# Autodesk Inventor assembly: basicLift
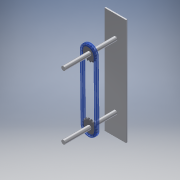
[picture p0: Inventor's stored thumbnail of the model, 180x180]
Saved by Autodesk Inventor 2016 SP1 (Build 200210100, 210)
## iProperties
Created: 2016-02-01
Part Number: basicLift
Document SubType Name: Assembly
Designer: steele
Mass: 210.898 g
Surface Area: 537.048 cm^2
Volume: 77.5037 cm^3
Density: 2.72113 g/cm^3
Author: steele
## Documents named in this file (4)
- C:\snobotics\CAD-Development\robSteele\SnoBotics2016\2016-01-31-Lift\basicLift.iam
- C:\snobotics\CAD-Development\robSteele\SnoBotics2016\2016-01-31-Lift\basicLiftPlate.ipt
- C:\snobotics\CAD-Development\robSteele\SnoBotics2016\2016-01-31-Lift\basicLeftAxel.ipt
- C:\snobotics\CAD-Development\robSteele\SnoBotics2016\2016-01-31-Lift\basicLift\Design Accelerator\Chain Drive1.iam
## Components (4 placed, 3 different names)
1. basicLiftPlate:1 — Insert:1, Insert:2
2. basicLeftAxel:1 — Insert:1
3. basicLeftAxel:2 — Insert:2
4. Chain Drive:1 [sub-assembly]
## Relationships (2: Insert 2)
- Insert:1: basicLiftPlate:1 ↔ basicLeftAxel:1
- Insert:2: basicLiftPlate:1 ↔ basicLeftAxel:2
